# Autodesk Inventor assembly: Anglerfish_bonne_mamman_m12large_v0
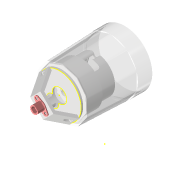
[picture p0: Inventor's stored thumbnail of the model, 180x180]
Saved by Autodesk Inventor 2022 (Build 260153000, 153)
## iProperties
Created: 2022-04-02
Part Number: Anglerfish_bonne_mamman_m12large_v0
Document SubType Name: Assembly
Designer: Prakash Lab
Author: Prakash Lab
## Documents named in this file (14)
- C:\Users\UC2\Documents\GitHub\Matchboxscope\INVENTOR\Anglerfish_bonne_mamman_m12large_v0.iam
- C:\Users\UC2\Documents\GitHub\Matchboxscope\INVENTOR\00_ESP3-CAM.iam
- C:\Users\UC2\Documents\GitHub\Matchboxscope\INVENTOR\00_Powerbank.ipt
- C:\Users\diederichbenedict\Documents\Inventor\Content Center Files\R2022\de-DE\DIN 912\DIN 912 - M3 x 0.5 x 25 x 18.ipt
- C:\Users\UC2\Documents\GitHub\Matchboxscope\INVENTOR\00_bonne_maman_jar.ipt
- C:\Users\UC2\Documents\GitHub\Matchboxscope\INVENTOR\Anglerfish_Jar_Adapterplate_v1.ipt
- C:\Users\UC2\Documents\GitHub\Matchboxscope\INVENTOR\Anglerfish_bottom_v0.ipt
- C:\Users\UC2\Documents\GitHub\Matchboxscope\INVENTOR\Matchboxscope_M12_Lensadapter_v0.ipt
- C:\Users\UC2\Documents\GitHub\Matchboxscope\INVENTOR\Anglerfish_Lightplate_Tosslink.ipt
- C:\Users\UC2\Documents\GitHub\Matchboxscope\INVENTOR\Importierte Komponenten\00_toslink_launcher_v3\00_toslink_launcher_v3.ipt
- C:\Users\UC2\Documents\GitHub\Matchboxscope\INVENTOR\Anglerfish_Lightplate_Tislinkbridge.ipt
- C:\Users\UC2\Documents\GitHub\Matchboxscope\INVENTOR\Anglerfish_middle2_m12VCMLens_large_v2.ipt
- C:\Users\UC2\Documents\GitHub\Matchboxscope\INVENTOR\00_CCTV_M12_VCM_large.ipt
- C:\Users\UC2\Documents\GitHub\Matchboxscope\INVENTOR\Anglerfish_spacer8mm_bottom_v0.ipt
## Components (15 placed, 13 different names)
1. 00_bonne_maman_jar:1 — Winkel:2, Passend:5, Fluchtend:2, Winkel:3, Passend:7, Winkel:4
2. DIN 912 - ersetzt durch DIN EN ISO 4762 M3 x 25:5
3. DIN 912 - ersetzt durch DIN EN ISO 4762 M3 x 25:7
4. DIN 912 - ersetzt durch DIN EN ISO 4762 M3 x 25:8
5. 00_toslink_launcher_v3:1 — Einfügen:11, Einfügen:12
6. Anglerfish_Lightplate_Tislinkbridge:1 — Einfügen:10, Einfügen:11, Einfügen:12
7. Anglerfish_Lightplate_Tosslink:1 — Einfügen:9, Einfügen:10
8. Anglerfish_Jar_Adapterplate_v1:1 — Passend:6, Passend:7, Einfügen:4, Fluchtend:3, Einfügen:9
9. Anglerfish_middle2_m12VCMLens_large_v2:1 — Einfügen:1, Passend:8, Einfügen:4, Winkel:4, Einfügen:5, Einfügen:6
10. 00_CCTV_M12_VCM_large:1 — Einfügen:1, Passend:8, Einfügen:3, Winkel:5
11. Matchboxscope_M12_Lensadapter_v0:1 — Einfügen:3, Passend:9
12. 00_Powerbank:1
13. 00_ESP3-CAM:1 [sub-assembly] — Passend:9, Fluchtend:3, Winkel:5
14. Anglerfish_bottom_v0:1 — Einfügen:7, Einfügen:8
15. Anglerfish_spacer8mm_bottom_v0:1 — Einfügen:5, Einfügen:6, Einfügen:7, Einfügen:8
## Relationships (22: Insert 11, Mate 5, Angle 4, Flush 2)
- Winkel:2 [Angle] (0 deg): 00_bonne_maman_jar:1
- Passend:5 [Mate]: 00_bonne_maman_jar:1
- Fluchtend:2 [Flush]: 00_bonne_maman_jar:1
- Winkel:3 [Angle] (0 deg): 00_bonne_maman_jar:1
- Passend:6 [Mate]: Anglerfish_Jar_Adapterplate_v1:1
- Passend:7 [Mate]: 00_bonne_maman_jar:1 ↔ Anglerfish_Jar_Adapterplate_v1:1
- Einfügen:1 [Insert]: Anglerfish_middle2_m12VCMLens_large_v2:1 ↔ 00_CCTV_M12_VCM_large:1
- Passend:8 [Mate]: Anglerfish_middle2_m12VCMLens_large_v2:1 ↔ 00_CCTV_M12_VCM_large:1
- Einfügen:3 [Insert] (-2 mm): 00_CCTV_M12_VCM_large:1 ↔ Matchboxscope_M12_Lensadapter_v0:1
- Einfügen:4 [Insert] (13 mm): Anglerfish_Jar_Adapterplate_v1:1 ↔ Anglerfish_middle2_m12VCMLens_large_v2:1
- Winkel:4 [Angle] (0 deg): 00_bonne_maman_jar:1 ↔ Anglerfish_middle2_m12VCMLens_large_v2:1
- Einfügen:5 [Insert]: Anglerfish_middle2_m12VCMLens_large_v2:1 ↔ Anglerfish_spacer8mm_bottom_v0:1
- Einfügen:6 [Insert]: Anglerfish_middle2_m12VCMLens_large_v2:1 ↔ Anglerfish_spacer8mm_bottom_v0:1
- Einfügen:7 [Insert]: Anglerfish_bottom_v0:1 ↔ Anglerfish_spacer8mm_bottom_v0:1
- Einfügen:8 [Insert]: Anglerfish_bottom_v0:1 ↔ Anglerfish_spacer8mm_bottom_v0:1
- Passend:9 [Mate]: Matchboxscope_M12_Lensadapter_v0:1 ↔ 00_ESP3-CAM:1
- Fluchtend:3 [Flush] (14 mm): Anglerfish_Jar_Adapterplate_v1:1 ↔ 00_ESP3-CAM:1
- Winkel:5 [Angle] (0 deg): 00_CCTV_M12_VCM_large:1 ↔ 00_ESP3-CAM:1
- Einfügen:9 [Insert] (4 mm): Anglerfish_Lightplate_Tosslink:1 ↔ Anglerfish_Jar_Adapterplate_v1:1
- Einfügen:10 [Insert]: Anglerfish_Lightplate_Tislinkbridge:1 ↔ Anglerfish_Lightplate_Tosslink:1
- Einfügen:11 [Insert]: 00_toslink_launcher_v3:1 ↔ Anglerfish_Lightplate_Tislinkbridge:1
- Einfügen:12 [Insert]: 00_toslink_launcher_v3:1 ↔ Anglerfish_Lightplate_Tislinkbridge:1
